# Autodesk Inventor assembly: Thumb_assembly
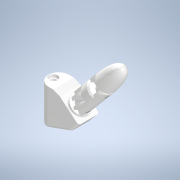
[picture p0: Inventor's stored thumbnail of the model, 180x180]
Saved by Autodesk Inventor 2022 (Build 260153000, 153)
## iProperties
Created: 2023-01-15
Part Number: Thumb_assembly
Document SubType Name: Assembly
Designer: 48735
Author: 48735
## Documents named in this file (5)
- C:\Users\48735\Desktop\Robot_hand_CAD\OSTATECZNA WERSJA\Thumb_assembly.iam
- C:\Users\48735\Desktop\Robot_hand_CAD\OSTATECZNA WERSJA\Main_part_thumb.ipt
- C:\Users\48735\Desktop\Robot_hand_CAD\OSTATECZNA WERSJA\Thumb_1.ipt
- C:\Users\48735\Desktop\Robot_hand_CAD\OSTATECZNA WERSJA\Thumb_2.ipt
- C:\Users\48735\Desktop\Robot_hand_CAD\OSTATECZNA WERSJA\Spring_thumb.ipt
## Components (7 placed, 4 different names)
1. Main_part_thumb:1 — Rotational:1, Rotational:5, Rigid:2
2. Thumb_1:1 — Rotational:1, Rotational:2
3. Thumb_2:1 — Rotational:2, Rotational:3, Rotational:4
4. Spring_thumb:1 — Rotational:4
5. Spring_thumb:2 — Rotational:3
6. Spring_thumb:3 — Rotational:5
7. Spring_thumb:4 — Rigid:2
## Relationships (6: RevoluteJoint 5, WeldJoint 1)
- Rotational:1 [RevoluteJoint]: Main_part_thumb:1 ↔ Thumb_1:1
- Rotational:2 [RevoluteJoint]: Thumb_1:1 ↔ Thumb_2:1
- Rotational:3 [RevoluteJoint]: Thumb_2:1 ↔ Spring_thumb:2
- Rotational:4 [RevoluteJoint] (3 mm): Thumb_2:1 ↔ Spring_thumb:1
- Rotational:5 [RevoluteJoint]: Main_part_thumb:1 ↔ Spring_thumb:3
- Rigid:2 [WeldJoint] (3 mm): Main_part_thumb:1 ↔ Spring_thumb:4
